# Autodesk Inventor assembly: Zespół1
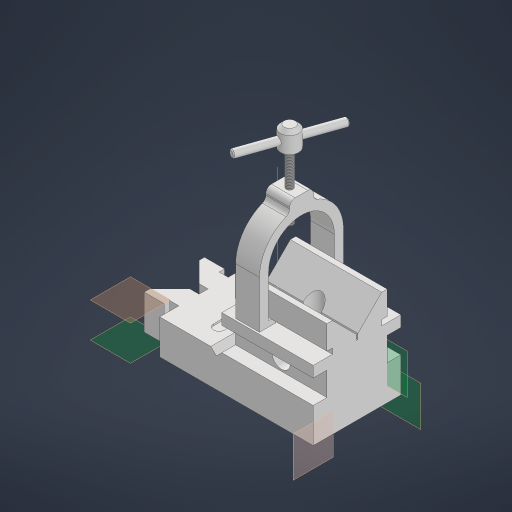
[picture p0: Inventor's stored thumbnail of the model, 512x512]
Saved by Autodesk Inventor 2023 (Build 270158000, 158)
## iProperties
Created: 2023-05-11
Part Number: Zespół1
Document SubType Name: Assembly
Designer: Adam
Author: Adam
## Documents named in this file (5)
- C:\Users\pryst\Desktop\KoNaR\Warsztaty\Mechanika\Projekty\Adam_Prystupa\Zespół1.iam
- C:\Users\pryst\Desktop\KoNaR\Warsztaty\Mechanika\Projekty\Adam_Prystupa\Część30.ipt
- C:\Users\pryst\Desktop\KoNaR\Warsztaty\Mechanika\Projekty\Adam_Prystupa\Część27.ipt
- C:\Users\pryst\Desktop\KoNaR\Warsztaty\Mechanika\Projekty\Adam_Prystupa\Część28.ipt
- C:\Users\pryst\Desktop\KoNaR\Warsztaty\Mechanika\Projekty\Adam_Prystupa\Część29.ipt
## Components (4 placed, 4 different names)
1. Część30:1 — przesuwne:1
2. Część27:1 — przesuwne:1, Zestawiające:1, Obrotowe:1
3. Część28:1 — Zestawiające:2, Zestawiające:3
4. Część29:1 — Zestawiające:1, Zestawiające:2, Zestawiające:3, Obrotowe:1
## Relationships (5: Mate 3, TranslationJoint 1, RevoluteJoint 1)
- przesuwne:1 [TranslationJoint] (0.5 mm): Część30:1 ↔ Część27:1
- Zestawiające:1 [Mate]: Część27:1 ↔ Część29:1
- Zestawiające:2 [Mate]: Część28:1 ↔ Część29:1
- Zestawiające:3 [Mate]: Część28:1 ↔ Część29:1
- Obrotowe:1 [RevoluteJoint]: Część27:1 ↔ Część29:1
